# Autodesk Inventor assembly: Sorting Assembly
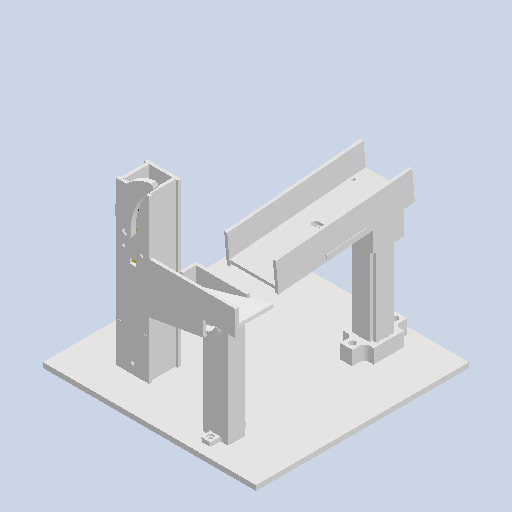
[picture p0: Inventor's stored thumbnail of the model, 512x512]
Saved by Autodesk Inventor 2025.4 (Build 294407000, 407)
## iProperties
Created: 2026-04-06
Part Number: Sorting Assembly
Document SubType Name: Assembly
Designer: lenovo
Author: lenovo
## Documents named in this file (18)
- F:\ASU Engineering\Year.2 ( 25-26 )\Spring\Basics Of Mechatronics\Project\Mechanisms\Shooting Mechanism\Shooting Assembly.iam
- F:\ASU Engineering\Year.2 ( 25-26 )\Spring\Basics Of Mechatronics\Project\Mechanisms\Shooting Mechanism\Base.ipt
- F:\ASU Engineering\Year.2 ( 25-26 )\Spring\Basics Of Mechatronics\Project\Mechanisms\Shooting Mechanism\Inclined Ramp.ipt
- F:\ASU Engineering\Year.2 ( 25-26 )\Spring\Basics Of Mechatronics\Project\Mechanisms\Shooting Mechanism\Motor Fixation .1.ipt
- F:\ASU Engineering\Year.2 ( 25-26 )\Spring\Basics Of Mechatronics\Project\Mechanisms\Shooting Mechanism\Motor Fixation .2.ipt
- F:\ASU Engineering\Year.2 ( 25-26 )\Spring\Basics Of Mechatronics\Project\Mechanisms\Shooting Mechanism\Ramp Side Wall.ipt
- F:\ASU Engineering\Year.2 ( 25-26 )\Spring\Basics Of Mechatronics\Project\Mechanisms\Shooting Mechanism\Path.ipt
- F:\ASU Engineering\Year.2 ( 25-26 )\Spring\Basics Of Mechatronics\Project\Mechanisms\Shooting Mechanism\Path Side Wall.ipt
- F:\ASU Engineering\Year.2 ( 25-26 )\Spring\Basics Of Mechatronics\Project\Mechanisms\Shooting Mechanism\Shooting Arm.ipt
- F:\ASU Engineering\Year.2 ( 25-26 )\Spring\Basics Of Mechatronics\Project\Mechanisms\Shooting Mechanism\Lower Path Fixation Shooting.ipt
- F:\ASU Engineering\Year.2 ( 25-26 )\Spring\Basics Of Mechatronics\Project\Mechanisms\Shooting Mechanism\Path Holder Shooting.ipt
- F:\ASU Engineering\Year.2 ( 25-26 )\Spring\Basics Of Mechatronics\Project\Mechanisms\Shooting Mechanism\Upper Path Fixation Shooting.ipt
- F:\ASU Engineering\Year.2 ( 25-26 )\Spring\Basics Of Mechatronics\Project\Mechanisms\Shooting Mechanism\IR Sensor\IR Sensor\IR Sensor.ipt
- F:\ASU Engineering\Year.2 ( 25-26 )\Spring\Basics Of Mechatronics\Project\Mechanisms\Shooting Mechanism\Motor Fixation .1 FV.ipt
- F:\ASU Engineering\Year.2 ( 25-26 )\Spring\Basics Of Mechatronics\Project\Mechanisms\Sorting Mechanism\DC Gear Motor Single Shaft\DC Gear Motor Single Shaft\DC Gear Motor Single Shaft.ipt
- F:\ASU Engineering\Year.2 ( 25-26 )\Spring\Basics Of Mechatronics\Project\Mechanisms\Shooting Mechanism\wall extension.ipt
- F:\ASU Engineering\Year.2 ( 25-26 )\Spring\Basics Of Mechatronics\Project\Mechanisms\Shooting Mechanism\ramp extension.ipt
- F:\ASU Engineering\Year.2 ( 25-26 )\Spring\Basics Of Mechatronics\Project\Mechanisms\Shooting Mechanism\Limit_Switch\Limit_Switch\Limit_Switch.ipt
## Components (23 placed, 17 different names)
1. Base:1 — Mate:1, Flush:4, Mate:12, Mate:29, Mate:30, Mate:31, Mate:55, Mate:56, Mate:63, Mate:69, Mate:82, Mate:83
2. Inclined Ramp:1 — Mate:1, Flush:4, Mate:13, Flush:7, Flush:8, Mate:14, Flush:9, Flush:10, Flush:30, Mate:55, Mate:56, Mate:78
3. Motor Fixation .1:2 — Mate:8, Mate:12, Mate:60, Mate:61, Mate:69, Mate:80
4. Motor Fixation .2:1 — Mate:80, Mate:81, Mate:82
5. Motor Fixation .2:2 — Mate:8, Mate:60, Mate:61, Mate:63, Mate:64, Mate:65, Mate:66, Flush:38
6. Ramp Side Wall:2 — Mate:13, Flush:7, Flush:8
7. Ramp Side Wall:3 — Mate:14, Flush:9, Flush:10, Mate:76, Flush:39, Flush:40
8. Path:1 — Mate:32, Mate:33, Mate:34, Mate:35, Flush:37, Mate:36, Mate:37, Mate:38
9. Path Side Wall:1 — Mate:34, Mate:35, Flush:37, Mate:39
10. Path Side Wall:2 — Mate:37, Mate:38, Mate:39
11. Shooting Arm:1 — Flush:30, Mate:75
12. Lower Path Fixation Shooting:1 — Mate:29, Mate:30, Mate:31, Mate:40, Mate:41, Mate:42, Mate:43, Mate:44, Mate:45, Mate:46, Mate:47, Mate:48, Mate:49, Mate:50, Mate:51
13. Upper Path Fixation Shooting:1 — Mate:32, Mate:33, Mate:36, Mate:52, Mate:53, Mate:54, Mate:70, Mate:71, Mate:72
14. Path Holder Shooting:1 — Mate:46, Mate:47, Mate:48, Mate:52, Mate:53, Mate:54
15. Path Holder Shooting:2 — Mate:49, Mate:50, Mate:51
16. Path Holder Shooting:3 — Mate:43, Mate:44, Mate:45
17. Path Holder Shooting:4 — Mate:40, Mate:41, Mate:42
18. IR Sensor:1 — Mate:70, Mate:71, Mate:72
19. Motor Fixation .1 FV:1 — Mate:64, Mate:65, Mate:66, Mate:73, Mate:74, Mate:79, Mate:81, Mate:83, Mate:84, Mate:85, Flush:41
20. DC Gear Motor Single Shaft:1 — Mate:73, Mate:74, Flush:38, Mate:75, Mate:79
21. wall extension:1 — Mate:76, Flush:39, Flush:40, Mate:77
22. ramp extension:1 — Mate:77, Mate:78
23. Limit_Switch:1 — Mate:84, Mate:85, Flush:41
## Relationships (67: Mate 56, Flush 11)
- Mate:1: Base:1 ↔ Inclined Ramp:1
- Flush:4 (10 mm): Base:1 ↔ Inclined Ramp:1
- Mate:8: Motor Fixation .1:2 ↔ Motor Fixation .2:2
- Mate:12: Base:1 ↔ Motor Fixation .1:2
- Mate:13: Inclined Ramp:1 ↔ Ramp Side Wall:2
- Flush:7: Inclined Ramp:1 ↔ Ramp Side Wall:2
- Flush:8: Inclined Ramp:1 ↔ Ramp Side Wall:2
- Mate:14: Inclined Ramp:1 ↔ Ramp Side Wall:3
- Flush:9: Inclined Ramp:1 ↔ Ramp Side Wall:3
- Flush:10: Inclined Ramp:1 ↔ Ramp Side Wall:3
- Flush:30: Inclined Ramp:1 ↔ Shooting Arm:1
- Mate:29: Base:1 ↔ Lower Path Fixation Shooting:1
- Mate:30: Base:1 ↔ Lower Path Fixation Shooting:1
- Mate:31: Base:1 ↔ Lower Path Fixation Shooting:1
- Mate:32: Path:1 ↔ Upper Path Fixation Shooting:1
- Mate:33: Path:1 ↔ Upper Path Fixation Shooting:1
- Mate:34: Path:1 ↔ Path Side Wall:1
- Mate:35: Path:1 ↔ Path Side Wall:1
- Flush:37: Path:1 ↔ Path Side Wall:1
- Mate:36: Path:1 ↔ Upper Path Fixation Shooting:1
- Mate:37: Path:1 ↔ Path Side Wall:2
- Mate:38: Path:1 ↔ Path Side Wall:2
- Mate:39: Path Side Wall:1 ↔ Path Side Wall:2
- Mate:40: Lower Path Fixation Shooting:1 ↔ Path Holder Shooting:4
- Mate:41: Lower Path Fixation Shooting:1 ↔ Path Holder Shooting:4
- Mate:42: Lower Path Fixation Shooting:1 ↔ Path Holder Shooting:4
- Mate:43: Lower Path Fixation Shooting:1 ↔ Path Holder Shooting:3
- Mate:44: Lower Path Fixation Shooting:1 ↔ Path Holder Shooting:3
- Mate:45: Lower Path Fixation Shooting:1 ↔ Path Holder Shooting:3
- Mate:46: Lower Path Fixation Shooting:1 ↔ Path Holder Shooting:1
- Mate:47: Lower Path Fixation Shooting:1 ↔ Path Holder Shooting:1
- Mate:48: Lower Path Fixation Shooting:1 ↔ Path Holder Shooting:1
- Mate:49: Lower Path Fixation Shooting:1 ↔ Path Holder Shooting:2
- Mate:50: Lower Path Fixation Shooting:1 ↔ Path Holder Shooting:2
- Mate:51: Lower Path Fixation Shooting:1 ↔ Path Holder Shooting:2
- Mate:52: Upper Path Fixation Shooting:1 ↔ Path Holder Shooting:1
- Mate:53: Upper Path Fixation Shooting:1 ↔ Path Holder Shooting:1
- Mate:54: Upper Path Fixation Shooting:1 ↔ Path Holder Shooting:1
- Mate:55: Base:1 ↔ Inclined Ramp:1
- Mate:56: Base:1 ↔ Inclined Ramp:1
- Mate:60: Motor Fixation .1:2 ↔ Motor Fixation .2:2
- Mate:61: Motor Fixation .1:2 ↔ Motor Fixation .2:2
- Mate:63: Base:1 ↔ Motor Fixation .2:2
- Mate:64: Motor Fixation .2:2 ↔ Motor Fixation .1 FV:1
- Mate:65: Motor Fixation .2:2 ↔ Motor Fixation .1 FV:1
- Mate:66: Motor Fixation .2:2 ↔ Motor Fixation .1 FV:1
- Mate:69: Base:1 ↔ Motor Fixation .1:2
- Mate:70: Upper Path Fixation Shooting:1 ↔ IR Sensor:1
- Mate:71: Upper Path Fixation Shooting:1 ↔ IR Sensor:1
- Mate:72: Upper Path Fixation Shooting:1 ↔ IR Sensor:1
- Mate:73: Motor Fixation .1 FV:1 ↔ DC Gear Motor Single Shaft:1
- Mate:74: Motor Fixation .1 FV:1 ↔ DC Gear Motor Single Shaft:1
- Flush:38: Motor Fixation .2:2 ↔ DC Gear Motor Single Shaft:1
- Mate:75: Shooting Arm:1 ↔ DC Gear Motor Single Shaft:1
- Mate:76: Ramp Side Wall:3 ↔ wall extension:1
- Flush:39: Ramp Side Wall:3 ↔ wall extension:1
- Flush:40: Ramp Side Wall:3 ↔ wall extension:1
- Mate:77: wall extension:1 ↔ ramp extension:1
- Mate:78: Inclined Ramp:1 ↔ ramp extension:1
- Mate:79: Motor Fixation .1 FV:1 ↔ DC Gear Motor Single Shaft:1
- Mate:80: Motor Fixation .1:2 ↔ Motor Fixation .2:1
- Mate:81: Motor Fixation .2:1 ↔ Motor Fixation .1 FV:1
- Mate:82: Base:1 ↔ Motor Fixation .2:1
- Mate:83: Base:1 ↔ Motor Fixation .1 FV:1
- Mate:84: Motor Fixation .1 FV:1 ↔ Limit_Switch:1
- Mate:85: Motor Fixation .1 FV:1 ↔ Limit_Switch:1
- Flush:41 (-2 mm): Motor Fixation .1 FV:1 ↔ Limit_Switch:1
